# Autodesk Inventor assembly: forkBaseWithWormGearAndLock
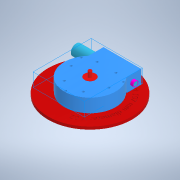
[picture p0: Inventor's stored thumbnail of the model, 180x180]
Saved by Autodesk Inventor 2022.2 (Build 262287010, 287A)
## iProperties
Created: 2020-11-22
Part Number: forkBaseWithWormGearAndLock
Document SubType Name: Assembly
Designer: robst
Author: robst
## Documents named in this file (11)
- C:\git\CAD-Development\robSteele\ShapeWays\TelescopeProjects\TelescopeMountNov2020\forkBaseWithWormGearAndLock.iam
- C:\git\CAD-Development\robSteele\ShapeWays\TelescopeProjects\TelescopeMountNov2020\baseSupport.ipt
- C:\git\CAD-Development\robSteele\ShapeWays\TelescopeProjects\TelescopeMount\forkMountForDecTripV01\Design Accelerator\Worm Gears5.iam
- C:\git\CAD-Development\robSteele\ShapeWays\TelescopeProjects\TelescopeMountNov2020\1_2x2x3_16-hexBearing.ipt
- C:\git\CAD-Development\robSteele\ShapeWays\TelescopeProjects\TelescopeMountNov2020\baseSupportCover.ipt
- c:\git\CAD-MfgResources\McMaster-Carr\Compression Spring\9657K512_COMPRESSION SPRING.ipt
- C:\git\CAD-Development\robSteele\ShapeWays\TelescopeProjects\TelescopeMountNov2020\3_8x7_5-inchHexShaft.ipt
- C:\git\CAD-Development\robSteele\ShapeWays\TelescopeProjects\TelescopeMountNov2020\3_8x3_4x3_4-hexBearing.ipt
- C:\git\CAD-Development\robSteele\ShapeWays\TelescopeProjects\TelescopeMountNov2020\3_8x3_4x3_4-hexBearingEndCap.ipt
- C:\git\CAD-Development\robSteele\ShapeWays\TelescopeProjects\TelescopeMountNov2020\gearLock1_00inchHexHole.ipt
- C:\git\CAD-Development\robSteele\ShapeWays\TelescopeProjects\TelescopeMountNov2020\1x8mmx1_1-inchHexShaft.ipt
## Components (10 placed, 10 different names)
1. baseSupport:1 — Insert:1, Insert:3, Mate:1, Flush:1, Flush:2, Insert:9, Insert:10
2. 3_8x7_5-inchHexShaft:1 — Insert:1, Insert:2
3. 3_8x3_4x3_4-hexBearing:1 — Insert:2
4. 3_8x3_4x3_4-hexBearingEndCap:1 — Insert:3
5. 1x8mmx1_1-inchHexShaft:1 — Insert:9
6. Worm Gears:1 [sub-assembly] — Insert:10, Mate:2, Mate:3
7. 1_2x2x3_16-hexBearing:1 — Insert:8
8. gearLock1_00inchHexHole:1 — Insert:8, Mate:2, Mate:3
9. baseSupportCover:1 — Mate:1, Flush:1, Flush:2
10. 9657K512_COMPRESSION SPRING:1
## Relationships (11: Insert 6, Mate 3, Flush 2)
- Insert:1: baseSupport:1 ↔ 3_8x7_5-inchHexShaft:1
- Insert:2: 3_8x7_5-inchHexShaft:1 ↔ 3_8x3_4x3_4-hexBearing:1
- Insert:3: baseSupport:1 ↔ 3_8x3_4x3_4-hexBearingEndCap:1
- Insert:8: 1_2x2x3_16-hexBearing:1 ↔ gearLock1_00inchHexHole:1
- Mate:1: baseSupport:1 ↔ baseSupportCover:1
- Flush:1: baseSupport:1 ↔ baseSupportCover:1
- Flush:2: baseSupport:1 ↔ baseSupportCover:1
- Insert:9: baseSupport:1 ↔ 1x8mmx1_1-inchHexShaft:1
- Insert:10: baseSupport:1 ↔ Worm Gears:1
- Mate:2: Worm Gears:1 ↔ gearLock1_00inchHexHole:1
- Mate:3: Worm Gears:1 ↔ gearLock1_00inchHexHole:1
